# Autodesk Inventor assembly: Prop
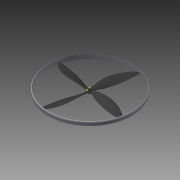
[picture p0: Inventor's stored thumbnail of the model, 180x180]
Saved by Autodesk Inventor 2015 (Build 190159000, 159)
## iProperties
Created: 2016-03-22
Part Number: Prop
Document SubType Name: Assembly
Designer: 839364
Author: 839364
## Documents named in this file (3)
- C:\Users\839364\Desktop\Drone\3D Models\Project\Prop.iam
- C:\Users\839364\Desktop\Drone\3D Models\Project\10x4.7.ipt
- C:\Users\839364\Desktop\Drone\3D Models\Project\Prop_Ring.ipt
## Components (3 placed, 2 different names)
1. 10x4.7:1 — Flush:1, Insert:1, Angle:1, Insert:2
2. 10x4.7:2 — Flush:1, Insert:1, Angle:1
3. Prop_Ring:1 — Insert:2
## Relationships (4: Insert 2, Flush 1, Angle 1)
- Flush:1: 10x4.7:1 ↔ 10x4.7:2
- Insert:1: 10x4.7:1 ↔ 10x4.7:2
- Angle:1 (90 deg): 10x4.7:1 ↔ 10x4.7:2
- Insert:2 (-6.35 mm): 10x4.7:1 ↔ Prop_Ring:1
